# Autodesk Inventor assembly: 8-mecanum-left-with-roller with hub
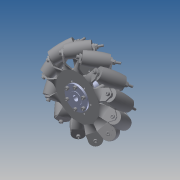
[picture p0: Inventor's stored thumbnail of the model, 180x180]
Saved by Autodesk Inventor 2014 SP1 (Build 180222100, 222)
## iProperties
Created: 2014-01-16
Part Number: 8-mecanum-left-with-roller with hub
Document SubType Name: Assembly
Designer: Pradhan Alexander
Author: Unknown
Title: //Amserv/amserver/AndyMark/Products/Wheel Mecanum/8 Mecanum Wheel/8 mecanum left with roller.stp
Organization: Unknown
Description: Unknown
Sending System: Unknown
Preprocessor: XStep 1.0
Author: Pradhan Alexander
## Documents named in this file (10)
- \\STUCLUSTER\Shared\MHS\Technology\Holliday B\Group Projects\Robotics\CAD Team\CAD Team 2014\Chassis 2014\8-mecanum-left-with-roller with hub.iam
- \\STUCLUSTER\Shared\MHS\Technology\Holliday B\Group Projects\Robotics\CAD Team\CAD Team 2014\Chassis 2014\Imported Components\8-mecanum-left-with-roller\#10 LockNut.ipt
- \\STUCLUSTER\Shared\MHS\Technology\Holliday B\Group Projects\Robotics\CAD Team\CAD Team 2014\Chassis 2014\Imported Components\8-mecanum-left-with-roller\Middle Axle.ipt
- \\STUCLUSTER\Shared\MHS\Technology\Holliday B\Group Projects\Robotics\CAD Team\CAD Team 2014\Chassis 2014\Imported Components\8-mecanum-left-with-roller\MBC Bushing MU04TH04.ipt
- \\STUCLUSTER\Shared\MHS\Technology\Holliday B\Group Projects\Robotics\CAD Team\CAD Team 2014\Chassis 2014\Imported Components\8-mecanum-left-with-roller\washer.ipt
- \\STUCLUSTER\Shared\MHS\Technology\Holliday B\Group Projects\Robotics\CAD Team\CAD Team 2014\Chassis 2014\Imported Components\8-mecanum-left-with-roller\SHCS 10-32x3_SHCS 10-32x3.ipt
- \\STUCLUSTER\Shared\MHS\Technology\Holliday B\Group Projects\Robotics\CAD Team\CAD Team 2014\Chassis 2014\Imported Components\8-mecanum-left-with-roller\Mid Roller III.ipt
- \\STUCLUSTER\Shared\MHS\Technology\Holliday B\Group Projects\Robotics\CAD Team\CAD Team 2014\Chassis 2014\Imported Components\8-mecanum-left-with-roller\8 Mecanum Plate Left.ipt
- \\STUCLUSTER\Shared\MHS\Technology\Holliday B\Group Projects\Robotics\CAD Team\CAD Team 2014\Chassis 2014\Imported Components\8-mecanum-left-with-roller\Spacer5.ipt
- \\STUCLUSTER\Shared\MHS\Technology\Holliday B\Group Projects\Robotics\CAD Team\CAD Team 2014\Chassis 2014\Imported Components\am-0077a-500 Key Hub r2\am-0077a-500 Key Hub r2.ipt
## Components (118 placed, 9 different names)
1. #10 LockNut
2. #10 LockNut:1
3. #10 LockNut:2
4. #10 LockNut:3 — Insert:12
5. #10 LockNut:4 — Insert:16
6. #10 LockNut:5
7. #10 LockNut:6
8. #10 LockNut:7
9. #10 LockNut:8 — Insert:11
10. #10 LockNut:9
11. #10 LockNut:10 — Insert:15
12. #10 LockNut:11
13. #10 LockNut:12
14. #10 LockNut:13 — Insert:13
15. #10 LockNut:14
16. #10 LockNut:15 — Insert:14
17. #10 LockNut:16
18. #10 LockNut:17
19. Middle Axle
20. Middle Axle:1
21. Middle Axle:2
22. Middle Axle:3
23. Middle Axle:4
24. Middle Axle:5
25. Middle Axle:6
26. Middle Axle:7
27. Middle Axle:8
28. Middle Axle:9
29. Middle Axle:10
30. Middle Axle:11
31. MBC Bushing MU04TH04
32. MBC Bushing MU04TH04:1
33. MBC Bushing MU04TH04:2
34. MBC Bushing MU04TH04:3
35. MBC Bushing MU04TH04:4
36. MBC Bushing MU04TH04:5
37. MBC Bushing MU04TH04:6
38. MBC Bushing MU04TH04:7
39. MBC Bushing MU04TH04:8
40. MBC Bushing MU04TH04:9
41. MBC Bushing MU04TH04:10
42. MBC Bushing MU04TH04:11
43. MBC Bushing MU04TH04:12
44. MBC Bushing MU04TH04:13
45. MBC Bushing MU04TH04:14
46. MBC Bushing MU04TH04:15
47. MBC Bushing MU04TH04:16
48. MBC Bushing MU04TH04:17
49. MBC Bushing MU04TH04:18
50. MBC Bushing MU04TH04:19
51. MBC Bushing MU04TH04:20
52. MBC Bushing MU04TH04:21
53. MBC Bushing MU04TH04:22
54. MBC Bushing MU04TH04:23
55. washer
56. washer:1
57. washer:2
58. washer:3
59. washer:4
60. washer:5
61. washer:6
62. washer:7
63. washer:8
64. washer:9
65. washer:10
66. washer:11
67. washer:12
68. washer:13
69. washer:14
70. washer:15
71. washer:16
72. washer:17
73. washer:18
74. washer:19
75. washer:20
76. washer:21
77. washer:22
78. washer:23
79. SHCS 10-32x3_SHCS 10-32x3 — Insert:10
80. SHCS 10-32x3_SHCS 10-32x3:1
81. SHCS 10-32x3_SHCS 10-32x3:2
82. SHCS 10-32x3_SHCS 10-32x3:3
83. SHCS 10-32x3_SHCS 10-32x3:4 — Insert:9
84. SHCS 10-32x3_SHCS 10-32x3:5 — Insert:6
85. SHCS 10-32x3_SHCS 10-32x3:6
86. SHCS 10-32x3_SHCS 10-32x3:7
87. SHCS 10-32x3_SHCS 10-32x3:8
88. SHCS 10-32x3_SHCS 10-32x3:9
89. SHCS 10-32x3_SHCS 10-32x3:10 — Insert:8
90. SHCS 10-32x3_SHCS 10-32x3:11
91. SHCS 10-32x3_SHCS 10-32x3:12
92. SHCS 10-32x3_SHCS 10-32x3:13 — Insert:5
93. SHCS 10-32x3_SHCS 10-32x3:14
94. SHCS 10-32x3_SHCS 10-32x3:15
95. SHCS 10-32x3_SHCS 10-32x3:16
96. SHCS 10-32x3_SHCS 10-32x3:17 — Insert:7
97. Mid Roller III
98. Mid Roller III:1
99. Mid Roller III:2
100. Mid Roller III:3
101. Mid Roller III:4
102. Mid Roller III:5
103. Mid Roller III:6
104. Mid Roller III:7
105. Mid Roller III:8
106. Mid Roller III:9
107. Mid Roller III:10
108. Mid Roller III:11
109. 8 Mecanum Plate Left — Insert:1, Insert:3
110. 8 Mecanum Plate Left:1 — Insert:2, Insert:4
111. Spacer5
112. Spacer5:1
113. Spacer5:2
114. Spacer5:3
115. Spacer5:4
116. Spacer5:5
117. am-0077a-500 Key Hub r2:1 — Insert:1, Insert:3, Insert:5, Insert:6, Insert:7, Insert:8, Insert:9, Insert:10
118. am-0077a-500 Key Hub r2:2 — Insert:2, Insert:4, Insert:11, Insert:12, Insert:13, Insert:14, Insert:15, Insert:16
## Relationships (16: Insert 16)
- Insert:1: 8 Mecanum Plate Left ↔ am-0077a-500 Key Hub r2:1
- Insert:2: 8 Mecanum Plate Left:1 ↔ am-0077a-500 Key Hub r2:2
- Insert:3: 8 Mecanum Plate Left ↔ am-0077a-500 Key Hub r2:1
- Insert:4: 8 Mecanum Plate Left:1 ↔ am-0077a-500 Key Hub r2:2
- Insert:5: SHCS 10-32x3_SHCS 10-32x3:13 ↔ am-0077a-500 Key Hub r2:1
- Insert:6: SHCS 10-32x3_SHCS 10-32x3:5 ↔ am-0077a-500 Key Hub r2:1
- Insert:7: SHCS 10-32x3_SHCS 10-32x3:17 ↔ am-0077a-500 Key Hub r2:1
- Insert:8: SHCS 10-32x3_SHCS 10-32x3:10 ↔ am-0077a-500 Key Hub r2:1
- Insert:9: SHCS 10-32x3_SHCS 10-32x3:4 ↔ am-0077a-500 Key Hub r2:1
- Insert:10: SHCS 10-32x3_SHCS 10-32x3 ↔ am-0077a-500 Key Hub r2:1
- Insert:11: #10 LockNut:8 ↔ am-0077a-500 Key Hub r2:2
- Insert:12: #10 LockNut:3 ↔ am-0077a-500 Key Hub r2:2
- Insert:13: #10 LockNut:13 ↔ am-0077a-500 Key Hub r2:2
- Insert:14: #10 LockNut:15 ↔ am-0077a-500 Key Hub r2:2
- Insert:15: #10 LockNut:10 ↔ am-0077a-500 Key Hub r2:2
- Insert:16: #10 LockNut:4 ↔ am-0077a-500 Key Hub r2:2
